# Autodesk Inventor assembly: power-distribution-power-distribution
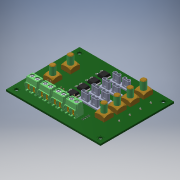
[picture p0: Inventor's stored thumbnail of the model, 180x180]
Saved by Autodesk Inventor 2019.4 (Build 234330000, 330)
## iProperties
Company: A Company
Created: 2020-08-04
Part Number: power-distribution-power-distribution
Description: KiCad electronic assembly
Document SubType Name: Assembly
Designer: Johansson
Authority: Unknown
Sending System: KiCad to STEP converter
Preprocessor: Open CASCADE STEP processor 6.9
Title: power-distribution.step
Author: An Author
## Documents named in this file (9)
- D:\Dropbox\Dokument\Projekt\Elita\Electrical system\Highside-Powerdistribution\hardware\cad\power-distribution\power-distribution-power-distribution.iam
- D:\Dropbox\Dokument\Projekt\Elita\Electrical system\Highside-Powerdistribution\hardware\cad\power-distribution\power-distribution-PinHeader_1x02_P2.54mm_Vertical.iam
- D:\Dropbox\Dokument\Projekt\Elita\Electrical system\Highside-Powerdistribution\hardware\cad\power-distribution\power-distribution-TO-252-2.iam
- D:\Dropbox\Dokument\Projekt\Elita\Electrical system\Highside-Powerdistribution\hardware\cad\power-distribution\power-distribution-R_0603_1608Metric.iam
- D:\Dropbox\Dokument\Projekt\Elita\Electrical system\Highside-Powerdistribution\hardware\cad\power-distribution\power-distribution-M5_7461383_rev1.iam
- D:\Dropbox\Dokument\Projekt\Elita\Electrical system\Highside-Powerdistribution\hardware\cad\power-distribution\power-distribution-LED_0603_1608Metric.iam
- D:\Dropbox\Dokument\Projekt\Elita\Electrical system\Highside-Powerdistribution\hardware\cad\power-distribution\power-distribution-keystone-PN3522-2.iam
- D:\Dropbox\Dokument\Projekt\Elita\Electrical system\Highside-Powerdistribution\hardware\cad\power-distribution\power-distribution-COMPOUND_1.ipt
- D:\Dropbox\Dokument\Projekt\Elita\Electrical system\Highside-Powerdistribution\hardware\cad\power-distribution\Phoenix_pxc_1935161_04_PT-1-5-2-5-0-H_3D.ipt
## Components (34 placed, 31 different names)
1. 2 [sub-assembly]
2. 3 [sub-assembly]
3. 4 [sub-assembly]
4. 6 [sub-assembly]
5. 7 [sub-assembly]
6. 8 [sub-assembly]
7. 9 [sub-assembly]
8. 11 [sub-assembly]
9. 12 [sub-assembly]
10. 13 [sub-assembly]
11. 14 [sub-assembly]
12. 16 [sub-assembly]
13. 17 [sub-assembly]
14. 19 [sub-assembly]
15. 20 [sub-assembly]
16. 21 [sub-assembly]
17. 22 [sub-assembly]
18. 23 [sub-assembly]
19. 24 [sub-assembly]
20. 25 [sub-assembly]
21. 26 [sub-assembly]
22. 27 [sub-assembly]
23. 28 [sub-assembly]
24. 29 [sub-assembly]
25. 30 [sub-assembly]
26. 32 [sub-assembly]
27. 33 [sub-assembly]
28. 34 [sub-assembly]
29. 35 [sub-assembly]
30. 36 — Mate:1, Mate:2, Mate:3
31. Phoenix_pxc_1935161_04_PT-1-5-2-5-0-H_3D:1 — Mate:1, Mate:2, Mate:3
32. Phoenix_pxc_1935161_04_PT-1-5-2-5-0-H_3D:2
33. Phoenix_pxc_1935161_04_PT-1-5-2-5-0-H_3D:3
34. Phoenix_pxc_1935161_04_PT-1-5-2-5-0-H_3D:4
## Component patterns: (4 elements, first: Phoenix_pxc_1935161_04_PT-1-5-2-5-0-H_3D:1)
## Relationships (3: Mate 3)
- Mate:1: 36 ↔ Phoenix_pxc_1935161_04_PT-1-5-2-5-0-H_3D:1
- Mate:2: 36 ↔ Phoenix_pxc_1935161_04_PT-1-5-2-5-0-H_3D:1
- Mate:3: 36 ↔ Phoenix_pxc_1935161_04_PT-1-5-2-5-0-H_3D:1
